# Autodesk Inventor assembly: wheal
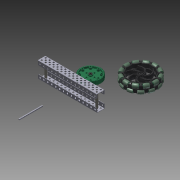
[picture p0: Inventor's stored thumbnail of the model, 180x180]
Saved by Autodesk Inventor 2015 (Build 190159000, 159)
## iProperties
Created: 2015-09-05
Part Number: wheal
Document SubType Name: Assembly
Designer: myps3_000
Author: myps3_000
## Documents named in this file (6)
- C:\Users\myps3_000\Desktop\dev\vex\custome\wheal.iam
- C:\Users\myps3_000\Desktop\dev\vex\Metal\C-Channels\C-Channel 1x2x1x15.ipt
- C:\Users\myps3_000\Desktop\dev\vex\Standoffs & Couplers\Standoff 2.00''.ipt
- C:\Users\myps3_000\Desktop\dev\vex\Drive Shafts\Drive Shaft 3''.ipt
- C:\Users\myps3_000\Desktop\dev\vex\Wheels\4'' Omni-Directional Wheel.iam
- C:\Users\myps3_000\Desktop\dev\vex\Spur Gears\High Strength 60-tooth Gear-Square Insert.iam
## Components (7 placed, 5 different names)
1. C-Channel 1x2x1x15:1 — Insert:1, Insert:2
2. C-Channel 1x2x1x15:2 — Insert:3
3. Standoff 2.00'':1 — Insert:2
4. Standoff 2.00'':2 — Insert:1, Insert:3
5. Drive Shaft 3'':1
6. 4'' Omni-Directional Wheel:1 [sub-assembly]
7. High Strength 60-tooth Gear-Square Insert:1 [sub-assembly]
## Relationships (3: Insert 3)
- Insert:1: C-Channel 1x2x1x15:1 ↔ Standoff 2.00'':2
- Insert:2: C-Channel 1x2x1x15:1 ↔ Standoff 2.00'':1
- Insert:3: C-Channel 1x2x1x15:2 ↔ Standoff 2.00'':2
